# Autodesk Inventor assembly: Knee_pitch_shim_basis
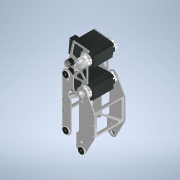
[picture p0: Inventor's stored thumbnail of the model, 180x180]
Saved by Autodesk Inventor 2020 (Build 240168000, 168)
## iProperties
Created: 2021-11-14
Part Number: Knee_pitch_shim_basis
Document SubType Name: Assembly
Designer: Masato Kubotera
Author: Masato Kubotera
## Documents named in this file (4)
- C:\Users\Masato\Documents\Inventor\CIT Brains_Inventor\OpenPlatform_ver3_0\Shim\Knee_pitch_shim_basis.iam
- C:\Users\Masato\Documents\Inventor\CIT Brains_Inventor\OpenPlatform_ver3_0\LowerBody\Knee\Knee.iam
- C:\Users\Masato\Documents\Inventor\CIT Brains_Inventor\OpenPlatform_ver3_0\LowerBody\Link\BackLink.iam
- C:\Users\Masato\Documents\Inventor\CIT Brains_Inventor\OpenPlatform_ver3_0\LowerBody\Link\FrontLink.iam
## Components (3 placed, 3 different names)
1. Knee:1 [sub-assembly] — 挿入:1, 挿入:2, 角度:1
2. BackLink:1 [sub-assembly] — 挿入:1, 角度:2
3. FrontLink:1 [sub-assembly] — 挿入:2, 角度:1, 角度:2
## Relationships (4: Insert 2, Angle 2)
- 挿入:1 [Insert]: Knee:1 ↔ BackLink:1
- 挿入:2 [Insert]: Knee:1 ↔ FrontLink:1
- 角度:1 [Angle] (0 deg): Knee:1 ↔ FrontLink:1
- 角度:2 [Angle] (0 deg): BackLink:1 ↔ FrontLink:1
